# Autodesk Inventor assembly: y-Max Endstop for 4040 - Assembly
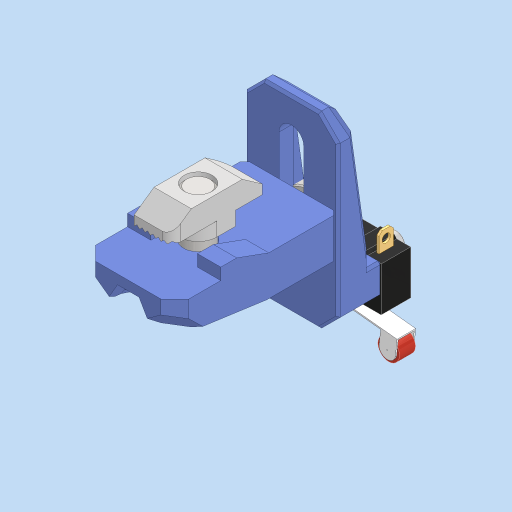
[picture p0: Inventor's stored thumbnail of the model, 512x512]
Saved by Autodesk Inventor 2023.2 (Build 272271000, 271)
## iProperties
Created: 2023-11-28
Part Number: y-Max Endstop for 4040 - Assembly
Document SubType Name: Assembly
Designer: Nils Bade
Author: Nils Bade
## Documents named in this file (9)
- C:\Users\nilsb\Documents\Inventor\Projektarbeit-Bade\RatRig_Bade\y-Max Endstop for 4040 - Assembly.iam
- C:\Users\nilsb\Documents\Inventor\Projektarbeit-Bade\RatRig_modified\y-Max Endstop Block for 4040.ipt
- C:\Users\nilsb\Documents\Inventor\Projektarbeit-Bade\RatRig_modified\T-NUT - DropIn 4040 SERIES - M6.ipt
- C:\Users\nilsb\Documents\Inventor\Projektarbeit-Bade\Schrauben\Cap Head Screw M6x12 v2.ipt
- C:\Users\nilsb\Documents\Inventor\Projektarbeit-Bade\Schrauben\Cap Head Screw M5x12 v2.ipt
- C:\Users\nilsb\Documents\Inventor\Projektarbeit-Bade\RatRig_Standards\Hex Locking Nut - M5 v2.ipt
- C:\Users\nilsb\Documents\Inventor\Projektarbeit-Bade\RatRig_modified\y-Max Endstop Slider for 4040.ipt
- C:\Users\nilsb\Documents\Inventor\Projektarbeit-Bade\RatRig_modified\NO-NC Limit Switch.ipt
- C:\Users\nilsb\Documents\Inventor\Projektarbeit-Bade\Schrauben\Cap Head Screw M2x10 - DIN912.ipt
## Components (9 placed, 8 different names)
1. y-Max Endstop Block for 4040:1 — Passend:1, Passend:2, Winkel:1, Passend:3, Passend:4, Passend:5, Winkel:2, Passend:6, Winkel:3, Passend:10
2. T-NUT - DROP IN TYPE FOR 40 SERIES - M6:1 — Passend:1, Passend:2, Winkel:1
3. Cap Head Screw M6x12 v2:1 — Passend:3, Passend:4
4. Cap Head Screw M5x12 v2:1 — Passend:7, Passend:8, Passend:9
5. Hex Locking Nut - M5 v2:1 — Passend:9, Winkel:3, Passend:10
6. y-Max Endstop Slider for 4040:1 — Passend:5, Winkel:2, Passend:6, Passend:7, Passend:8, Passend:11, Passend:12, Passend:13
7. NO-NC Limit Switch:1 — Passend:11, Passend:12, Passend:13, Passend:14, Passend:15, Passend:16, Passend:17
8. Cap Head Screw M2x10 - DIN912:1 — Passend:14, Passend:17
9. Cap Head Screw M2x10 - DIN912:2 — Passend:15, Passend:16
## Relationships (20: Mate 17, Angle 3)
- Passend:1 [Mate]: y-Max Endstop Block for 4040:1 ↔ T-NUT - DROP IN TYPE FOR 40 SERIES - M6:1
- Passend:2 [Mate] (5.5 mm): y-Max Endstop Block for 4040:1 ↔ T-NUT - DROP IN TYPE FOR 40 SERIES - M6:1
- Winkel:1 [Angle] (0 deg): y-Max Endstop Block for 4040:1 ↔ T-NUT - DROP IN TYPE FOR 40 SERIES - M6:1
- Passend:3 [Mate]: y-Max Endstop Block for 4040:1 ↔ Cap Head Screw M6x12 v2:1
- Passend:4 [Mate]: y-Max Endstop Block for 4040:1 ↔ Cap Head Screw M6x12 v2:1
- Passend:5 [Mate]: y-Max Endstop Block for 4040:1 ↔ y-Max Endstop Slider for 4040:1
- Winkel:2 [Angle] (0 deg): y-Max Endstop Block for 4040:1 ↔ y-Max Endstop Slider for 4040:1
- Passend:6 [Mate]: y-Max Endstop Block for 4040:1 ↔ y-Max Endstop Slider for 4040:1
- Passend:7 [Mate]: Cap Head Screw M5x12 v2:1 ↔ y-Max Endstop Slider for 4040:1
- Passend:8 [Mate]: Cap Head Screw M5x12 v2:1 ↔ y-Max Endstop Slider for 4040:1
- Passend:9 [Mate]: Cap Head Screw M5x12 v2:1 ↔ Hex Locking Nut - M5 v2:1
- Winkel:3 [Angle] (0 deg): y-Max Endstop Block for 4040:1 ↔ Hex Locking Nut - M5 v2:1
- Passend:10 [Mate]: y-Max Endstop Block for 4040:1 ↔ Hex Locking Nut - M5 v2:1
- Passend:11 [Mate]: y-Max Endstop Slider for 4040:1 ↔ NO-NC Limit Switch:1
- Passend:12 [Mate]: y-Max Endstop Slider for 4040:1 ↔ NO-NC Limit Switch:1
- Passend:13 [Mate]: y-Max Endstop Slider for 4040:1 ↔ NO-NC Limit Switch:1
- Passend:14 [Mate]: NO-NC Limit Switch:1 ↔ Cap Head Screw M2x10 - DIN912:1
- Passend:15 [Mate]: NO-NC Limit Switch:1 ↔ Cap Head Screw M2x10 - DIN912:2
- Passend:16 [Mate]: NO-NC Limit Switch:1 ↔ Cap Head Screw M2x10 - DIN912:2
- Passend:17 [Mate]: NO-NC Limit Switch:1 ↔ Cap Head Screw M2x10 - DIN912:1
